# Autodesk Inventor assembly: 전체조립
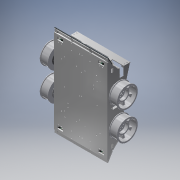
[picture p0: Inventor's stored thumbnail of the model, 180x180]
Saved by Autodesk Inventor 2017 (Build 210142000, 142)
## iProperties
Part Number: 전체조립
Material: 일반
Document SubType Name: Assembly
Designer: minom
Mass: 2106.19 g
Surface Area: 5683.51 cm^2
Volume: 937.335 cm^3
Density: 2.247 g/cm^3
Author: minom
## Documents named in this file (16)
- C:\Users\Minos\Documents\Inventor\Projects\2017 IRC Sumo Mino ver.2\전체조립.iam
- C:\Users\Minos\Documents\Inventor\Projects\2017 IRC Sumo Mino ver.2\밑판받침대조립품.iam
- C:\Users\Minos\Documents\Inventor\Projects\2017 IRC Sumo Mino ver.2\옆판베어링결합_오른쪽.iam
- C:\Users\Minos\Documents\Inventor\Projects\2017 IRC Sumo Mino ver.2\옆판베어링결합_왼쪽.iam
- C:\Users\Minos\Documents\Inventor\Projects\2017 IRC Sumo Mino ver.2\바퀴풀리결합_8PI.iam
- C:\Users\Minos\Documents\Inventor\Projects\2017 IRC Sumo Mino ver.2\베어링받침대결합.iam
- C:\Users\Minos\Documents\Inventor\Projects\2017 IRC Sumo Mino ver.2\바퀴풀리결합_10PI.iam
- C:\Users\Minos\Documents\Inventor\Projects\2017 IRC Sumo Mino ver.2\8060모터드라이브.ipt
- C:\Users\Minos\Documents\Inventor\Projects\2017 IRC Sumo Mino ver.2\대각선PSD받침대.ipt
- C:\Users\Minos\Documents\Inventor\Projects\2017 IRC Sumo Mino ver.2\앞뒷면PSD받침대_수정.ipt
- C:\Users\Minos\Documents\Inventor\Projects\2017 IRC Sumo Mino ver.2\CdS모듈.ipt
- C:\Users\Minos\Documents\Inventor\Projects\2017 IRC Sumo Mino ver.2\앞뒷판_위_수정.ipt
- C:\Users\Minos\Documents\Inventor\Projects\2017 IRC Sumo Mino ver.2\앞뒷판_중간.ipt
- C:\Users\Minos\Documents\Inventor\Projects\2017 IRC Sumo Mino ver.2\앞뒷판_밑.ipt
- C:\Users\Minos\Documents\Inventor\Projects\2017 IRC Sumo Mino ver.2\IR모듈.ipt
- C:\Users\Minos\Documents\Inventor\Projects\2017 IRC Sumo Mino ver.2\CAD 도면\칼팁.ipt
## Components (30 placed, 15 different names)
1. 밑판받침대조립품:1 [sub-assembly] — 메이트:1, 메이트:2, 메이트:42, 메이트:43, 메이트:44, 메이트:45, 메이트:46, 메이트:47, 메이트:48, 메이트:49, 메이트:51, 메이트:53, 메이트:62, 메이트:63, 메이트:74, 메이트:75, 메이트:76, 메이트:77, 메이트:82, 메이트:83, 메이트:84, 메이트:86, 메이트:87, 메이트:89, 메이트:90, 메이트:92, 메이트:93, 메이트:94, 메이트:95, 메이트:96, 메이트:98, 메이트:99, 메이트:100, 메이트:101, 메이트:102, 메이트:103, 메이트:104, 메이트:105, 메이트:106, 메이트:107, 메이트:108, 메이트:109, 메이트:110, 메이트:111, 메이트:112, 메이트:113, 메이트:114, 메이트:116, 메이트:118, 메이트:120, 메이트:122
2. 옆판베어링결합_오른쪽:1 [sub-assembly] — 메이트:43, 메이트:44, 메이트:45, 메이트:52, 메이트:56, 메이트:57, 메이트:61, 메이트:64, 플러쉬:1, 각도:1, 각도:4, 메이트:78, 메이트:79, 메이트:117, 메이트:119
3. 옆판베어링결합_왼쪽:1 [sub-assembly] — 메이트:46, 메이트:47, 메이트:48, 메이트:50, 메이트:54, 메이트:55, 메이트:59, 메이트:65, 플러쉬:2, 각도:2, 각도:3, 메이트:80, 메이트:81, 메이트:115, 메이트:121
4. 베어링받침대결합:2 [sub-assembly] — 메이트:42, 메이트:49, 메이트:50, 메이트:58
5. 베어링받침대결합:3 [sub-assembly] — 메이트:51, 메이트:52, 메이트:53, 메이트:60
6. 바퀴풀리결합_8PI:1 [sub-assembly] — 메이트:56, 메이트:57
7. 바퀴풀리결합_8PI:2 [sub-assembly] — 메이트:54, 메이트:55
8. 바퀴풀리결합_10PI:1 [sub-assembly] — 메이트:60, 메이트:61
9. 바퀴풀리결합_10PI:2 [sub-assembly] — 메이트:58, 메이트:59
10. 8060모터드라이브:1 — 메이트:62, 메이트:64, 플러쉬:1
11. 8060모터드라이브:2 — 메이트:63, 메이트:65, 플러쉬:2
12. 대각선PSD받침대:1 — 메이트:74, 각도:1, 메이트:78, 메이트:82, 메이트:91
13. 대각선PSD받침대:2 — 메이트:75, 각도:2, 메이트:81, 메이트:83
14. 대각선PSD받침대:3 — 메이트:77, 각도:3, 메이트:80, 메이트:84
15. 대각선PSD받침대:4 — 메이트:76, 각도:4, 메이트:79, 메이트:88
16. 앞뒷면PSD받침대_수정:1 — 메이트:87, 메이트:88, 메이트:89
17. 앞뒷면PSD받침대_수정:2 — 메이트:86, 메이트:90, 메이트:91
18. CdS모듈:1 — 메이트:93, 메이트:95, 플러쉬:3, 플러쉬:4
19. CdS모듈:2 — 메이트:92, 메이트:94, 플러쉬:5, 플러쉬:6
20. 앞뒷판_위_수정:1 — 메이트:99, 메이트:100, 메이트:101
21. 앞뒷판_위_수정:2 — 메이트:96, 메이트:98, 메이트:102
22. 앞뒷판_중간:1 — 메이트:103, 메이트:104, 메이트:105
23. 앞뒷판_중간:2 — 메이트:106, 메이트:107, 메이트:108
24. 앞뒷판_밑:1 — 메이트:109, 메이트:110, 메이트:111, 플러쉬:7
25. 앞뒷판_밑:2 — 메이트:112, 메이트:113, 메이트:114
26. IR모듈:1 — 플러쉬:4, 메이트:117, 메이트:118
27. IR모듈:2 — 플러쉬:3, 메이트:115, 메이트:116
28. IR모듈:3 — 플러쉬:5, 메이트:119, 메이트:120
29. IR모듈:4 — 플러쉬:6, 메이트:121, 메이트:122
30. 칼팁:1 — 플러쉬:7
## Relationships (84: Mate 73, Flush 7, Angle 4)
- 메이트:1 [Mate] (10 mm): 밑판받침대조립품:1
- 메이트:2 [Mate]: 밑판받침대조립품:1
- 메이트:42 [Mate] (0.1 mm): 밑판받침대조립품:1 ↔ 베어링받침대결합:2
- 메이트:43 [Mate]: 밑판받침대조립품:1 ↔ 옆판베어링결합_오른쪽:1
- 메이트:44 [Mate] (10 mm): 밑판받침대조립품:1 ↔ 옆판베어링결합_오른쪽:1
- 메이트:45 [Mate] (0.1 mm): 밑판받침대조립품:1 ↔ 옆판베어링결합_오른쪽:1
- 메이트:46 [Mate]: 밑판받침대조립품:1 ↔ 옆판베어링결합_왼쪽:1
- 메이트:47 [Mate] (0.1 mm): 밑판받침대조립품:1 ↔ 옆판베어링결합_왼쪽:1
- 메이트:48 [Mate] (10 mm): 밑판받침대조립품:1 ↔ 옆판베어링결합_왼쪽:1
- 메이트:49 [Mate]: 밑판받침대조립품:1 ↔ 베어링받침대결합:2
- 메이트:50 [Mate]: 옆판베어링결합_왼쪽:1 ↔ 베어링받침대결합:2
- 메이트:51 [Mate]: 밑판받침대조립품:1 ↔ 베어링받침대결합:3
- 메이트:52 [Mate]: 옆판베어링결합_오른쪽:1 ↔ 베어링받침대결합:3
- 메이트:53 [Mate] (0.1 mm): 밑판받침대조립품:1 ↔ 베어링받침대결합:3
- 메이트:54 [Mate] (2 mm): 옆판베어링결합_왼쪽:1 ↔ 바퀴풀리결합_8PI:2
- 메이트:55 [Mate]: 옆판베어링결합_왼쪽:1 ↔ 바퀴풀리결합_8PI:2
- 메이트:56 [Mate]: 옆판베어링결합_오른쪽:1 ↔ 바퀴풀리결합_8PI:1
- 메이트:57 [Mate] (2 mm): 옆판베어링결합_오른쪽:1 ↔ 바퀴풀리결합_8PI:1
- 메이트:58 [Mate]: 베어링받침대결합:2 ↔ 바퀴풀리결합_10PI:2
- 메이트:59 [Mate] (2 mm): 옆판베어링결합_왼쪽:1 ↔ 바퀴풀리결합_10PI:2
- 메이트:60 [Mate]: 베어링받침대결합:3 ↔ 바퀴풀리결합_10PI:1
- 메이트:61 [Mate] (2 mm): 옆판베어링결합_오른쪽:1 ↔ 바퀴풀리결합_10PI:1
- 메이트:62 [Mate] (50 mm): 밑판받침대조립품:1 ↔ 8060모터드라이브:1
- 메이트:63 [Mate] (50 mm): 밑판받침대조립품:1 ↔ 8060모터드라이브:2
- 메이트:64 [Mate] (25 mm): 옆판베어링결합_오른쪽:1 ↔ 8060모터드라이브:1
- 메이트:65 [Mate] (25 mm): 옆판베어링결합_왼쪽:1 ↔ 8060모터드라이브:2
- 플러쉬:1 [Flush] (32 mm): 옆판베어링결합_오른쪽:1 ↔ 8060모터드라이브:1
- 플러쉬:2 [Flush] (32 mm): 옆판베어링결합_왼쪽:1 ↔ 8060모터드라이브:2
- 메이트:74 [Mate]: 밑판받침대조립품:1 ↔ 대각선PSD받침대:1
- 메이트:75 [Mate]: 밑판받침대조립품:1 ↔ 대각선PSD받침대:2
- 메이트:76 [Mate]: 밑판받침대조립품:1 ↔ 대각선PSD받침대:4
- 메이트:77 [Mate]: 밑판받침대조립품:1 ↔ 대각선PSD받침대:3
- 각도:1 [Angle] (45 deg): 옆판베어링결합_오른쪽:1 ↔ 대각선PSD받침대:1
- 각도:2 [Angle] (315 deg): 옆판베어링결합_왼쪽:1 ↔ 대각선PSD받침대:2
- 각도:3 [Angle] (45 deg): 옆판베어링결합_왼쪽:1 ↔ 대각선PSD받침대:3
- 각도:4 [Angle] (315 deg): 옆판베어링결합_오른쪽:1 ↔ 대각선PSD받침대:4
- 메이트:78 [Mate] (4 mm): 옆판베어링결합_오른쪽:1 ↔ 대각선PSD받침대:1
- 메이트:79 [Mate] (4 mm): 옆판베어링결합_오른쪽:1 ↔ 대각선PSD받침대:4
- 메이트:80 [Mate] (4 mm): 옆판베어링결합_왼쪽:1 ↔ 대각선PSD받침대:3
- 메이트:81 [Mate] (4 mm): 옆판베어링결합_왼쪽:1 ↔ 대각선PSD받침대:2
- 메이트:82 [Mate] (4 mm): 밑판받침대조립품:1 ↔ 대각선PSD받침대:1
- 메이트:83 [Mate] (4 mm): 밑판받침대조립품:1 ↔ 대각선PSD받침대:2
- 메이트:84 [Mate] (4 mm): 밑판받침대조립품:1 ↔ 대각선PSD받침대:3
- 메이트:86 [Mate]: 밑판받침대조립품:1 ↔ 앞뒷면PSD받침대_수정:2
- 메이트:87 [Mate]: 밑판받침대조립품:1 ↔ 앞뒷면PSD받침대_수정:1
- 메이트:88 [Mate] (13 mm): 대각선PSD받침대:4 ↔ 앞뒷면PSD받침대_수정:1
- 메이트:89 [Mate] (21 mm): 밑판받침대조립품:1 ↔ 앞뒷면PSD받침대_수정:1
- 메이트:90 [Mate] (21 mm): 밑판받침대조립품:1 ↔ 앞뒷면PSD받침대_수정:2
- 메이트:91 [Mate] (13 mm): 대각선PSD받침대:1 ↔ 앞뒷면PSD받침대_수정:2
- 메이트:92 [Mate] (5 mm): 밑판받침대조립품:1 ↔ CdS모듈:2
- 메이트:93 [Mate] (5 mm): 밑판받침대조립품:1 ↔ CdS모듈:1
- 메이트:94 [Mate] (18.9 mm): 밑판받침대조립품:1 ↔ CdS모듈:2
- 메이트:95 [Mate] (18.9 mm): 밑판받침대조립품:1 ↔ CdS모듈:1
- 메이트:96 [Mate]: 밑판받침대조립품:1 ↔ 앞뒷판_위_수정:2
- 메이트:98 [Mate]: 밑판받침대조립품:1 ↔ 앞뒷판_위_수정:2
- 메이트:99 [Mate]: 밑판받침대조립품:1 ↔ 앞뒷판_위_수정:1
- 메이트:100 [Mate] (0.1 mm): 밑판받침대조립품:1 ↔ 앞뒷판_위_수정:1
- 메이트:101 [Mate]: 밑판받침대조립품:1 ↔ 앞뒷판_위_수정:1
- 메이트:102 [Mate] (0.1 mm): 밑판받침대조립품:1 ↔ 앞뒷판_위_수정:2
- 메이트:103 [Mate] (0.1 mm): 밑판받침대조립품:1 ↔ 앞뒷판_중간:1
- 메이트:104 [Mate]: 밑판받침대조립품:1 ↔ 앞뒷판_중간:1
- 메이트:105 [Mate]: 밑판받침대조립품:1 ↔ 앞뒷판_중간:1
- 메이트:106 [Mate]: 밑판받침대조립품:1 ↔ 앞뒷판_중간:2
- 메이트:107 [Mate] (0.1 mm): 밑판받침대조립품:1 ↔ 앞뒷판_중간:2
- 메이트:108 [Mate]: 밑판받침대조립품:1 ↔ 앞뒷판_중간:2
- 메이트:109 [Mate]: 밑판받침대조립품:1 ↔ 앞뒷판_밑:1
- 메이트:110 [Mate] (0.1 mm): 밑판받침대조립품:1 ↔ 앞뒷판_밑:1
- 메이트:111 [Mate]: 밑판받침대조립품:1 ↔ 앞뒷판_밑:1
- 메이트:112 [Mate]: 밑판받침대조립품:1 ↔ 앞뒷판_밑:2
- 메이트:113 [Mate] (0.1 mm): 밑판받침대조립품:1 ↔ 앞뒷판_밑:2
- 메이트:114 [Mate]: 밑판받침대조립품:1 ↔ 앞뒷판_밑:2
- 플러쉬:3 [Flush]: CdS모듈:1 ↔ IR모듈:2
- 메이트:115 [Mate] (3 mm): 옆판베어링결합_왼쪽:1 ↔ IR모듈:2
- 메이트:116 [Mate] (6 mm): 밑판받침대조립품:1 ↔ IR모듈:2
- 플러쉬:4 [Flush]: CdS모듈:1 ↔ IR모듈:1
- 메이트:117 [Mate] (3 mm): 옆판베어링결합_오른쪽:1 ↔ IR모듈:1
- 메이트:118 [Mate] (6 mm): 밑판받침대조립품:1 ↔ IR모듈:1
- 플러쉬:5 [Flush]: CdS모듈:2 ↔ IR모듈:3
- 메이트:119 [Mate] (3 mm): 옆판베어링결합_오른쪽:1 ↔ IR모듈:3
- 메이트:120 [Mate] (6 mm): 밑판받침대조립품:1 ↔ IR모듈:3
- 플러쉬:6 [Flush]: CdS모듈:2 ↔ IR모듈:4
- 메이트:121 [Mate] (3 mm): 옆판베어링결합_왼쪽:1 ↔ IR모듈:4
- 메이트:122 [Mate] (6 mm): 밑판받침대조립품:1 ↔ IR모듈:4
- 플러쉬:7 [Flush]: 앞뒷판_밑:1 ↔ 칼팁:1
